# Autodesk Inventor assembly: montagem centrifuga2
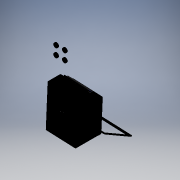
[picture p0: Inventor's stored thumbnail of the model, 180x180]
Saved by Autodesk Inventor 2019 (Build 230136000, 136)
## iProperties
Created: 2019-11-06
Part Number: montagem centrifuga2
Material: Genérico
Document SubType Name: Assembly
Designer: natha
Author: natha
## Documents named in this file (16)
- C:\Users\55119\Desktop\Final-20191204T124812Z-001\Final\montagem centrifuga2.iam
- C:\Users\55119\Desktop\Final-20191204T124812Z-001\Final\casenova.ipt
- C:\Users\55119\Desktop\Final-20191204T124812Z-001\Final\encaixe fonte.ipt
- C:\Users\55119\Desktop\Final-20191204T124812Z-001\Final\containment - Copia.ipt
- C:\Users\55119\Desktop\Final-20191204T124812Z-001\Final\tacometer_ct.ipt
- C:\Users\55119\Desktop\Final-20191204T124812Z-001\Final\motorMount.ipt
- C:\Users\55119\Desktop\Final-20191204T124812Z-001\Final\User Library-LCD-5.iam
- C:\Users\55119\Desktop\Final-20191204T124812Z-001\Final\tampa extra.ipt
- C:\Users\55119\Desktop\Final-20191204T124812Z-001\Final\chapaaço.ipt
- C:\Users\55119\Desktop\Final-20191204T124812Z-001\Final\Tech Makers-AK360_7000.iam
- C:\Users\55119\Desktop\Final-20191204T124812Z-001\Final\counter.0001.ipt
- C:\Users\55119\Desktop\Final-20191204T124812Z-001\Final\tampa acrilico.ipt
- C:\Users\55119\Desktop\Final-20191204T124812Z-001\Final\rotor.ipt
- C:\Users\55119\Desktop\Final-20191204T124812Z-001\Final\pé.ipt
- C:\Users\55119\Desktop\Final-20191204T124812Z-001\Final\painel lcd.ipt
- C:\Users\55119\Desktop\Final-20191204T124812Z-001\Final\suporte interno.ipt
## Components (15 placed, 15 different names)
1. casenova:1 — Cilíndrica:1, Plana:2, Coincidência:5, Coincidência:7, Coincidência:8, Coincidência:9, Coincidência:10, Coincidência:12, Coincidência:14, Coincidência:18, Coincidência:19, Coincidência:20, Cilíndrica:9, Cilíndrica:10, Coincidência:22, Coincidência:23
2. encaixe fonte:1 — Cilíndrica:1, Plana:2
3. containment - Copia:1 — Coincidência:14, Coincidência:15, Coincidência:18, Coincidência:19, Cilíndrica:6
4. tacometer_ct:1 — Tangente:1, Alinhamento:2
5. motorMount:1 — Coincidência:13, Cilíndrica:4, Alinhamento:1, Tangente:1, Alinhamento:2, Cilíndrica:6
6. User Library-LCD-5:1 [sub-assembly] — Coincidência:5
7. tampa extra:1 — Coincidência:7, Coincidência:8, Coincidência:9, Coincidência:15, Coincidência:17, Cilíndrica:5
8. chapaaço:1 — Coincidência:10, Coincidência:12, Coincidência:13, Coincidência:20
9. Tech Makers-AK360_7000:1 [sub-assembly] — Cilíndrica:4, Alinhamento:1, Coincidência:16, Cilíndrica:7, Cilíndrica:8, Cilíndrica:11
10. counter.0001:1 — Coincidência:16, Coincidência:21, Cilíndrica:8
11. tampa acrilico:1 — Coincidência:17, Cilíndrica:5
12. rotor:1 — Cilíndrica:7, Coincidência:21
13. pé:1
14. painel lcd:1 — Cilíndrica:9, Cilíndrica:10
15. suporte interno:1 — Coincidência:22, Cilíndrica:11, Coincidência:23
## Relationships (30: Mate 17, CylindricalJoint 9, Flush 2, PlanarJoint 1, Tangent 1)
- Cilíndrica:1 [CylindricalJoint]: casenova:1 ↔ encaixe fonte:1
- Plana:2: casenova:1 ↔ encaixe fonte:1
- Coincidência:5 [Mate]: casenova:1 ↔ User Library-LCD-5:1
- Coincidência:7 [Mate]: casenova:1 ↔ tampa extra:1
- Coincidência:8 [Mate]: casenova:1 ↔ tampa extra:1
- Coincidência:9 [Mate]: casenova:1 ↔ tampa extra:1
- Coincidência:10 [Mate]: casenova:1 ↔ chapaaço:1
- Coincidência:12 [Mate]: casenova:1 ↔ chapaaço:1
- Coincidência:13 [Mate]: motorMount:1 ↔ chapaaço:1
- Coincidência:14 [Mate] (1 mm): casenova:1 ↔ containment - Copia:1
- Coincidência:15 [Mate]: containment - Copia:1 ↔ tampa extra:1
- Cilíndrica:4 [CylindricalJoint]: motorMount:1 ↔ Tech Makers-AK360_7000:1
- Alinhamento:1 [Flush]: motorMount:1 ↔ Tech Makers-AK360_7000:1
- Coincidência:16 [Mate] (1 mm): Tech Makers-AK360_7000:1 ↔ counter.0001:1
- Tangente:1: tacometer_ct:1 ↔ motorMount:1
- Alinhamento:2 [Flush]: tacometer_ct:1 ↔ motorMount:1
- Coincidência:17 [Mate]: tampa extra:1 ↔ tampa acrilico:1
- Cilíndrica:5 [CylindricalJoint]: tampa extra:1 ↔ tampa acrilico:1
- Coincidência:18 [Mate] (1 mm): casenova:1 ↔ containment - Copia:1
- Coincidência:19 [Mate] (1 mm): casenova:1 ↔ containment - Copia:1
- Coincidência:20 [Mate] (10 mm): casenova:1 ↔ chapaaço:1
- Cilíndrica:6 [CylindricalJoint]: containment - Copia:1 ↔ motorMount:1
- Cilíndrica:7 [CylindricalJoint]: Tech Makers-AK360_7000:1 ↔ rotor:1
- Coincidência:21 [Mate]: counter.0001:1 ↔ rotor:1
- Cilíndrica:8 [CylindricalJoint]: Tech Makers-AK360_7000:1 ↔ counter.0001:1
- Cilíndrica:9 [CylindricalJoint]: casenova:1 ↔ painel lcd:1
- Cilíndrica:10 [CylindricalJoint]: casenova:1 ↔ painel lcd:1
- Coincidência:22 [Mate]: casenova:1 ↔ suporte interno:1
- Cilíndrica:11 [CylindricalJoint]: Tech Makers-AK360_7000:1 ↔ suporte interno:1
- Coincidência:23 [Mate] (1.5 mm): casenova:1 ↔ suporte interno:1
